# Autodesk Inventor assembly: MagneticEncoder V2
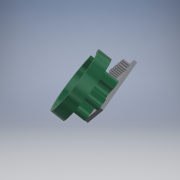
[picture p0: Inventor's stored thumbnail of the model, 180x180]
Saved by Autodesk Inventor 2019.1 (Build 231200000, 200)
## iProperties
Created: 2018-11-04
Part Number: MagneticEncoder V2
Material: Generisch
Document SubType Name: Assembly
Designer: JochenAlt
Author: JochenAlt
## Documents named in this file (5)
- D:\Projects\Ondine\CAD\Encoder\MagneticEncoder V2.iam
- D:\Projects\Ondine\CAD\Encoder\MagnetHolder.ipt
- D:\Projects\Ondine\CAD\Encoder\Magnet.ipt
- D:\Projects\Ondine\CAD\Encoder\AS5047D.ipt
- D:\Projects\Ondine\CAD\Encoder\AS5047DEnclosureV2.ipt
## Components (4 placed, 4 different names)
1. MagnetHolder:1 — Passend:6, Passend:7, Passend:21
2. Magnet:1 — Passend:6, Passend:7, Passend:18
3. AS5047D:1 — Passend:18, Passend:22, Passend:23
4. AS5047DEnclosureV2:1 — Passend:21, Passend:22, Passend:23
## Relationships (6: Mate 6)
- Passend:6 [Mate]: MagnetHolder:1 ↔ Magnet:1
- Passend:7 [Mate]: MagnetHolder:1 ↔ Magnet:1
- Passend:18 [Mate] (0.5 mm): Magnet:1 ↔ AS5047D:1
- Passend:21 [Mate]: MagnetHolder:1 ↔ AS5047DEnclosureV2:1
- Passend:22 [Mate]: AS5047D:1 ↔ AS5047DEnclosureV2:1
- Passend:23 [Mate]: AS5047D:1 ↔ AS5047DEnclosureV2:1
